# Autodesk Inventor assembly: stepstick+female adapter
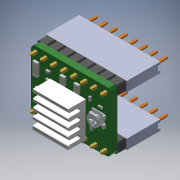
[picture p0: Inventor's stored thumbnail of the model, 180x180]
Saved by Autodesk Inventor 2018 (Build 220112000, 112)
## iProperties
Created: 2015-05-03
Part Number: stepstick+female adapter
Document SubType Name: Assembly
Designer: Gabriel Smolnycki
Sending System: SolidWorks 2013
Last Author: paolo
Last Saved: 2015-05-04
Author: Gabriel Smolnycki
## Documents named in this file (11)
- E:\planb\mechanics\V1INV\Electronics\Megatronics\stepstick+female adapter.iam
- E:\planb\mechanics\V1INV\Electronics\Megatronics\stepstick.ipt
- E:\planb\mechanics\V1INV\Electronics\Megatronics\0402CAP_CAP0402CAP.ipt
- E:\planb\mechanics\V1INV\Electronics\Megatronics\1206_CAP1206.ipt
- E:\planb\mechanics\V1INV\Electronics\Megatronics\QFN28ET_A4983.ipt
- E:\planb\mechanics\V1INV\Electronics\Megatronics\0402RES_RESISTOR0402RES.ipt
- E:\planb\mechanics\V1INV\Electronics\Megatronics\0805_RESISTOR.ipt
- E:\planb\mechanics\V1INV\Electronics\Megatronics\TRIMPOT3MM_TRIMPOTSMD.ipt
- E:\planb\mechanics\V1INV\Electronics\Megatronics\Pin header pitch 2.54mm(08 contacts).ipt
- E:\planb\mechanics\V1INV\Electronics\Megatronics\Heatsink For A4988.ipt
- E:\planb\mechanics\V1INV\Electronics\Megatronics\female_header.ipt
## Components (21 placed, 10 different names)
1. stepstick:1 — Flush:1, Flush:2
2. 0402CAP_CAP0402CAP:1
3. 0402CAP_CAP0402CAP:2
4. 0402CAP_CAP0402CAP:3
5. 0402CAP_CAP0402CAP:4
6. 0402CAP_CAP0402CAP:5
7. 0402CAP_CAP0402CAP:6
8. 1206_CAP1206:1
9. QFN28ET_A4983:1 — Mate:1
10. 0402RES_RESISTOR0402RES:1
11. 0402RES_RESISTOR0402RES:2
12. 0402RES_RESISTOR0402RES:3
13. 0402RES_RESISTOR0402RES:4
14. 0805_RESISTOR:1
15. 0805_RESISTOR:2
16. TRIMPOT3MM_TRIMPOTSMD:1
17. Pin header pitch 2.54mm(08 contacts):1
18. Pin header pitch 2.54mm(08 contacts):2
19. Heatsink For A4988:1 — Mate:1, Flush:1, Flush:2
20. female_header:1
21. female_header:2
## Relationships (3: Flush 2, Mate 1)
- Mate:1: QFN28ET_A4983:1 ↔ Heatsink For A4988:1
- Flush:1 (2.3 mm): stepstick:1 ↔ Heatsink For A4988:1
- Flush:2 (5 mm): stepstick:1 ↔ Heatsink For A4988:1
